# Autodesk Inventor assembly: Robot mrk3
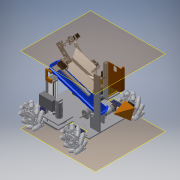
[picture p0: Inventor's stored thumbnail of the model, 180x180]
Saved by Autodesk Inventor 2019 (Build 230136000, 136)
## iProperties
Created: 2017-12-06
Part Number: Robot mrk3
Document SubType Name: Assembly
Designer: User
Author: User
## Documents named in this file (21)
- D:\robotics\Robot mrk2.iam
- D:\robotics\CAD\2017-18_CAD\Prototypes\Gen2PlatePart.ipt
- D:\robotics\CAD\2017-18_CAD\Prototypes\MecanumWheelFullForVexmotor.iam
- D:\robotics\CAD\COTSParts\Rev\REV-41-1300HexMotor.ipt
- D:\robotics\CAD\2017-18_CAD\Prototypes\MotorHolderA.ipt
- D:\robotics\CAD\2017-18_CAD\Prototypes\MotorHolderB.ipt
- D:\robotics\CAD\2018-19_CAD\Collection\SlidesPivotBracket.ipt
- D:\robotics\CAD\2018-19_CAD\lift\lift assembly\Lead Screw Prototype A.iam
- D:\robotics\CAD\2018-19_CAD\Collection\CollectionPost.ipt
- D:\robotics\CAD\2017-18_CAD\battery for holder.iam
- D:\robotics\CAD\2018-19_CAD\3d printer\MotoGPhoneHolder.ipt
- D:\robotics\CAD\COTSParts\Bosch Extrusion\Bosch 20x20 8.5inch.ipt
- D:\robotics\CAD\COTSParts\Motors\am-3102NeveRest20 (1).ipt
- D:\robotics\CAD\COTSParts\Actobotics\555 parts\555116ClampingMotorMount37mmBottomBore.ipt
- D:\robotics\CAD\2018-19_CAD\3d printer\marker pyramid.ipt
- D:\robotics\CAD\COTSParts\Rev\REV-31-1153RevHub.ipt
- D:\robotics\CAD\2018-19_CAD\Collection\sorterbucket.iam
- D:\robotics\CAD\2018-19_CAD\Collection\slide to axle bracet.ipt
- D:\robotics\CAD\2016-17_CAD\Lift2.iam
- D:\robotics\CAD\2018-19_CAD\marker release.iam
- D:\robotics\CAD\2018-19_CAD\bucket hlder.ipt
## Components (32 placed, 20 different names)
1. Gen2PlatePart:1 — Flush:36, Mate:34, Flush:37, Mate:37, Mate:38, Flush:42, Mate:41, Flush:48, Flush:51, Flush:53, Mate:59, Flush:58, Mate:64, Flush:59, Mate:67, Mate:68, Angle:5, Mate:69, Flush:60, Mate:73, Mate:74, Flush:61, Flush:62, Mate:75, Mate:77, Mate:78, Mate:80, Mate:81, Mate:84, Mate:85, Mate:89, Mate:91, Flush:93, Flush:94
2. MecanumWheelFullForVexmotor:1 [sub-assembly] — Insert:24, Rotation:2, Rotation:3
3. MecanumWheelFullForVexmotor:2 [sub-assembly] — Rotation:1, Mate:70, Mate:71, Mate:72
4. MecanumWheelFullForVexmotor:3 [sub-assembly] — Insert:23, Rotation:1, Rotation:3
5. REV-41-1300HexMotor:2 — Mate:24, Insert:23, Mate:50, Angle:4
6. REV-41-1300HexMotor:3 — Insert:24, Mate:46, Angle:3, Mate:47
7. REV-41-1300HexMotor:4 — Angle:1, Mate:65, Mate:66, Mate:70, Mate:71, Mate:72
8. MotorHolderA:1 — Mate:24, Flush:52, Mate:50, Angle:4, Mate:69, Flush:60
9. MotorHolderA:2 — Insert:25, Flush:48, Angle:2, Mate:74, Flush:62, Mate:79
10. MotorHolderB:1 — Mate:46, Angle:3, Mate:47, Flush:52, Mate:67, Mate:68, Angle:5
11. MotorHolderB:2 — Angle:1, Flush:51, Mate:65, Mate:66, Mate:73, Flush:61
12. REV-41-1300HexMotor:5 — Insert:25, Insert:26, Angle:2
13. MecanumWheelFullForVexmotor:4 [sub-assembly] — Insert:26, Rotation:2
14. SlidesPivotBracket:1 — Flush:64, Mate:81, Mate:82, Flush:65, Insert:27
15. SlidesPivotBracket:2 — Flush:64, Mate:82, Mate:84, Mate:89, Mate:90, Flush:72, Flush:74
16. Lead Screw Prototype A:1 [sub-assembly] — Mate:34, Flush:37, Flush:59
17. CollectionPost:1 — Flush:53, Mate:80, Flush:65
18. battery for holder:1 [sub-assembly] — Mate:37, Mate:38, Flush:42
19. MotoGPhoneHolder:1 — Mate:42, Mate:43, Flush:44
20. Bosch 20x20 8.5inch:1 — Mate:41, Mate:42, Mate:43, Flush:44, Flush:58, Mate:64
21. am-3102NeveRest20 (1):1 — Mate:52, Flush:54
22. am-3102NeveRest20 (1):2 — Mate:51, Flush:55
23. 555116ClampingMotorMount37mmBottomBore:1 — Mate:51, Flush:55, Mate:85, Mate:90, Flush:72, Flush:73
24. 555116ClampingMotorMount37mmBottomBore:2 — Mate:52, Flush:54, Mate:59, Flush:73, Flush:74
25. marker pyramid:2 — Mate:92, Mate:93
26. REV-31-1153RevHub:1 — Mate:75
27. REV-31-1153RevHub:2 — Mate:77, Mate:78, Mate:79
28. sorterbucket:1 [sub-assembly] — Mate:87, Flush:75, Flush:76, Flush:95
29. slide to axle bracet:1 — Insert:27, Mate:86, Flush:70, Flush:71
30. Lift2:1 [sub-assembly] — Mate:86, Flush:70, Flush:71, Mate:87, Flush:75, Flush:76, Mate:94, Flush:96
31. marker release:1 [sub-assembly] — Mate:91, Flush:93, Flush:94, Mate:92, Mate:93
32. bucket hlder:1 — Mate:94, Flush:95, Flush:96
## Relationships (83: Mate 41, Flush 29, Angle 5, Insert 5, RelateRotation 3)
- Mate:24: REV-41-1300HexMotor:2 ↔ MotorHolderA:1
- Angle:1 (180 deg): REV-41-1300HexMotor:4 ↔ MotorHolderB:2
- Insert:23: MecanumWheelFullForVexmotor:3 ↔ REV-41-1300HexMotor:2
- Insert:24: MecanumWheelFullForVexmotor:1 ↔ REV-41-1300HexMotor:3
- Insert:25: MotorHolderA:2 ↔ REV-41-1300HexMotor:5
- Insert:26: REV-41-1300HexMotor:5 ↔ MecanumWheelFullForVexmotor:4
- Rotation:1 [RelateRotation] (1 ul): MecanumWheelFullForVexmotor:2 ↔ MecanumWheelFullForVexmotor:3
- Rotation:2 [RelateRotation] (1 ul): MecanumWheelFullForVexmotor:1 ↔ MecanumWheelFullForVexmotor:4
- Rotation:3 [RelateRotation] (1 ul): MecanumWheelFullForVexmotor:1 ↔ MecanumWheelFullForVexmotor:3
- Flush:36 (360.0704 mm): Gen2PlatePart:1
- Mate:34: Gen2PlatePart:1 ↔ Lead Screw Prototype A:1
- Flush:37: Gen2PlatePart:1 ↔ Lead Screw Prototype A:1
- Mate:37: Gen2PlatePart:1 ↔ battery for holder:1
- Mate:38: Gen2PlatePart:1 ↔ battery for holder:1
- Flush:42: Gen2PlatePart:1 ↔ battery for holder:1
- Mate:41: Gen2PlatePart:1 ↔ Bosch 20x20 8.5inch:1
- Mate:42: MotoGPhoneHolder:1 ↔ Bosch 20x20 8.5inch:1
- Mate:43 (3.048 mm): MotoGPhoneHolder:1 ↔ Bosch 20x20 8.5inch:1
- Flush:44: MotoGPhoneHolder:1 ↔ Bosch 20x20 8.5inch:1
- Flush:48: Gen2PlatePart:1 ↔ MotorHolderA:2
- Angle:2 (180 deg): MotorHolderA:2 ↔ REV-41-1300HexMotor:5
- Mate:46: REV-41-1300HexMotor:3 ↔ MotorHolderB:1
- Angle:3 (180 deg): REV-41-1300HexMotor:3 ↔ MotorHolderB:1
- Mate:47: REV-41-1300HexMotor:3 ↔ MotorHolderB:1
- Flush:51: Gen2PlatePart:1 ↔ MotorHolderB:2
- Flush:52: MotorHolderA:1 ↔ MotorHolderB:1
- Mate:50: REV-41-1300HexMotor:2 ↔ MotorHolderA:1
- Angle:4 (180 deg): REV-41-1300HexMotor:2 ↔ MotorHolderA:1
- Flush:53: Gen2PlatePart:1 ↔ CollectionPost:1
- Mate:51: am-3102NeveRest20 (1):2 ↔ 555116ClampingMotorMount37mmBottomBore:1
- Mate:52: am-3102NeveRest20 (1):1 ↔ 555116ClampingMotorMount37mmBottomBore:2
- Flush:54: am-3102NeveRest20 (1):1 ↔ 555116ClampingMotorMount37mmBottomBore:2
- Flush:55: am-3102NeveRest20 (1):2 ↔ 555116ClampingMotorMount37mmBottomBore:1
- Mate:59: Gen2PlatePart:1 ↔ 555116ClampingMotorMount37mmBottomBore:2
- Flush:58: Gen2PlatePart:1 ↔ Bosch 20x20 8.5inch:1
- Mate:64 (-6.35 mm): Gen2PlatePart:1 ↔ Bosch 20x20 8.5inch:1
- Mate:65: REV-41-1300HexMotor:4 ↔ MotorHolderB:2
- Mate:66: REV-41-1300HexMotor:4 ↔ MotorHolderB:2
- Flush:59 (10.16 mm): Gen2PlatePart:1 ↔ Lead Screw Prototype A:1
- Mate:67: Gen2PlatePart:1 ↔ MotorHolderB:1
- Mate:68: Gen2PlatePart:1 ↔ MotorHolderB:1
- Angle:5 (0 deg): Gen2PlatePart:1 ↔ MotorHolderB:1
- Mate:69: Gen2PlatePart:1 ↔ MotorHolderA:1
- Flush:60: Gen2PlatePart:1 ↔ MotorHolderA:1
- Mate:70: MecanumWheelFullForVexmotor:2 ↔ REV-41-1300HexMotor:4
- Mate:71: MecanumWheelFullForVexmotor:2 ↔ REV-41-1300HexMotor:4
- Mate:72: MecanumWheelFullForVexmotor:2 ↔ REV-41-1300HexMotor:4
- Mate:73: Gen2PlatePart:1 ↔ MotorHolderB:2
- Mate:74: Gen2PlatePart:1 ↔ MotorHolderA:2
- Flush:61: Gen2PlatePart:1 ↔ MotorHolderB:2
- Flush:62: Gen2PlatePart:1 ↔ MotorHolderA:2
- Flush:63 (-457.2 mm)
- Mate:75: Gen2PlatePart:1 ↔ REV-31-1153RevHub:1
- Mate:77: Gen2PlatePart:1 ↔ REV-31-1153RevHub:2
- Mate:78: Gen2PlatePart:1 ↔ REV-31-1153RevHub:2
- Mate:79 (38.1 mm): MotorHolderA:2 ↔ REV-31-1153RevHub:2
- Mate:80: Gen2PlatePart:1 ↔ CollectionPost:1
- Flush:64: SlidesPivotBracket:1 ↔ SlidesPivotBracket:2
- Mate:81: Gen2PlatePart:1 ↔ SlidesPivotBracket:1
- Mate:82 (57.15 mm): SlidesPivotBracket:1 ↔ SlidesPivotBracket:2
- Flush:65: SlidesPivotBracket:1 ↔ CollectionPost:1
- Mate:84: Gen2PlatePart:1 ↔ SlidesPivotBracket:2
- Mate:85: Gen2PlatePart:1 ↔ 555116ClampingMotorMount37mmBottomBore:1
- Insert:27: SlidesPivotBracket:1 ↔ slide to axle bracet:1
- Mate:86: slide to axle bracet:1 ↔ Lift2:1
- Flush:70 (22.606 mm): slide to axle bracet:1 ↔ Lift2:1
- Flush:71 (-13.081 mm): slide to axle bracet:1 ↔ Lift2:1
- Mate:87 (12.7 mm): sorterbucket:1 ↔ Lift2:1
- Mate:89: Gen2PlatePart:1 ↔ SlidesPivotBracket:2
- Mate:90 (6.35 mm): SlidesPivotBracket:2 ↔ 555116ClampingMotorMount37mmBottomBore:1
- Flush:72 (-10.16 mm): SlidesPivotBracket:2 ↔ 555116ClampingMotorMount37mmBottomBore:1
- Flush:73 (45.72 mm): 555116ClampingMotorMount37mmBottomBore:1 ↔ 555116ClampingMotorMount37mmBottomBore:2
- Flush:74 (-71.12 mm): SlidesPivotBracket:2 ↔ 555116ClampingMotorMount37mmBottomBore:2
- Flush:75 (17.0815 mm): sorterbucket:1 ↔ Lift2:1
- Flush:76 (25.4 mm): sorterbucket:1 ↔ Lift2:1
- Mate:91 (12.7 mm): Gen2PlatePart:1 ↔ marker release:1
- Flush:93: Gen2PlatePart:1 ↔ marker release:1
- Flush:94 (-6.35 mm): Gen2PlatePart:1 ↔ marker release:1
- Mate:92: marker pyramid:2 ↔ marker release:1
- Mate:93: marker pyramid:2 ↔ marker release:1
- Mate:94: Lift2:1 ↔ bucket hlder:1
- Flush:95: sorterbucket:1 ↔ bucket hlder:1
- Flush:96 (14.986 mm): Lift2:1 ↔ bucket hlder:1
